# Autodesk Inventor assembly: RspCameraMia
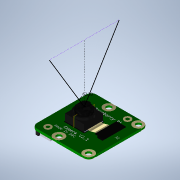
[picture p0: Inventor's stored thumbnail of the model, 180x180]
Saved by Autodesk Inventor 2020.3 (Build 243373000, 373)
## iProperties
Created: 2018-02-03
Part Number: RspCameraMia
Material: Genérico
Document SubType Name: Assembly
Designer: RafaX
Author: RafaX
## Documents named in this file (17)
- C:\Users\juanp\Desktop\Robocol\Nuevo EVA\Recursos\Pi Camera\RspCameraMia.iam
- C:\Users\juanp\Desktop\Robocol\Nuevo EVA\Recursos\Pi Camera\PicameraPCB.ipt
- C:\Users\juanp\Desktop\Robocol\Nuevo EVA\Recursos\Pi Camera\OVA5647_Housing.ipt
- C:\Users\juanp\Desktop\Robocol\Nuevo EVA\Recursos\Pi Camera\OVA5647_Lens_FOV.ipt
- C:\Users\juanp\Desktop\Robocol\Nuevo EVA\Recursos\Pi Camera\ribbon_cam.ipt
- C:\Users\juanp\Desktop\Robocol\Nuevo EVA\Recursos\Pi Camera\CCD.ipt
- C:\Users\juanp\Desktop\Robocol\Nuevo EVA\Recursos\Pi Camera\CAPC-0805-T0.75-BN.ipt
- C:\Users\juanp\Desktop\Robocol\Nuevo EVA\Recursos\Pi Camera\CAPC-0402-T0.55-BN.ipt
- C:\Users\juanp\Desktop\Robocol\Nuevo EVA\Recursos\Pi Camera\RESC-0402.ipt
- C:\Users\juanp\Desktop\Robocol\Nuevo EVA\Recursos\Pi Camera\RESC-0603.ipt
- C:\Users\juanp\Desktop\Robocol\Nuevo EVA\Recursos\Pi Camera\RESC-1210.ipt
- C:\Users\juanp\Desktop\Robocol\Nuevo EVA\Recursos\Pi Camera\c-1-1734248-5-e-raspberry_display.ipt
- C:\Users\juanp\Desktop\Robocol\Nuevo EVA\Recursos\Pi Camera\SOT23-5.ipt
- C:\Users\juanp\Desktop\Robocol\Nuevo EVA\Recursos\Pi Camera\KX7 SMD Quartz Crystal Resonator 3.2x2.5mm.ipt
- C:\Users\juanp\Desktop\Robocol\Nuevo EVA\Recursos\Pi Camera\70521906.iam
- C:\Users\juanp\Desktop\Robocol\Nuevo EVA\Recursos\Pi Camera\c6aaa.ipt
- C:\Users\juanp\Desktop\Robocol\Nuevo EVA\Recursos\Pi Camera\4pin_smd.ipt
## Components (33 placed, 16 different names)
1. PicameraPCB:1
2. OVA5647_Housing:1 — Flush:1
3. OVA5647_Lens_FOV:1
4. ribbon_cam:1
5. CCD:1
6. CAPC-0805-T0.75-BN:1
7. CAPC-0805-T0.75-BN:2
8. CAPC-0402-T0.55-BN:1
9. CAPC-0402-T0.55-BN:2
10. CAPC-0402-T0.55-BN:3
11. CAPC-0402-T0.55-BN:4
12. CAPC-0402-T0.55-BN:5
13. CAPC-0402-T0.55-BN:6
14. CAPC-0402-T0.55-BN:7
15. CAPC-0402-T0.55-BN:8
16. CAPC-0402-T0.55-BN:9
17. CAPC-0402-T0.55-BN:10
18. RESC-0402:1
19. RESC-0402:2
20. RESC-0402:5
21. RESC-0603:1
22. RESC-0603:2
23. RESC-1210:1
24. c-1-1734248-5-e-raspberry_display:1
25. SOT23-5:1
26. SOT23-5:2
27. SOT23-5:3
28. KX7 SMD Quartz Crystal Resonator 3.2x2.5mm:4
29. 70521906:1 [sub-assembly]
30. c6aaa:1
31. 4pin_smd:1
32. 4pin_smd:2
33. 4pin_smd:3
## Relationships (1: Flush 1)
- Flush:1: OVA5647_Housing:1
